# Autodesk Inventor assembly: Assembly2
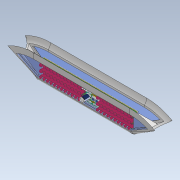
[picture p0: Inventor's stored thumbnail of the model, 180x180]
Saved by Autodesk Inventor 2021 (Build 250183000, 183)
## iProperties
Created: 2020-10-01
Part Number: Assembly2
Document SubType Name: Assembly
Designer: capta
Author: capta
## Documents named in this file (5)
- C:\Users\capta\OneDrive - Lehigh University\Formula SAE\Tractive Light\Assembly2.iam
- C:\Users\capta\OneDrive - Lehigh University\Formula SAE\Tractive Light\Tractive Light Enclosure 3.0.ipt
- C:\Users\capta\OneDrive - Lehigh University\Formula SAE\Tractive Light\Mount CAD\pcd stand in.ipt
- C:\Users\capta\OneDrive - Lehigh University\Formula SAE\Tractive Light\acrlyc 2.0.ipt
- C:\Users\capta\OneDrive - Lehigh University\Formula SAE\Tractive Light\PCB Assembly\Tractive PCB.iam
## Components (5 placed, 4 different names)
1. Tractive Light Enclosure 3.0:1 — Mate:1, Mate:2, Mate:3, Mate:4, Mate:5, Mate:6, Mate:7, Mate:8, Mate:9, Mate:10, Mate:11, Mate:12
2. pcd stand in:1 — Mate:1, Mate:2, Mate:3
3. acrlyc 2.0:1 — Mate:4, Mate:5, Mate:6
4. acrlyc 2.0:2 — Mate:7, Mate:8, Mate:9
5. Tractive PCB:1 [sub-assembly] — Mate:10, Mate:11, Mate:12
## Relationships (14: Mate 12, Flush 2)
- Mate:1: Tractive Light Enclosure 3.0:1 ↔ pcd stand in:1
- Mate:2 (0.381 mm): Tractive Light Enclosure 3.0:1 ↔ pcd stand in:1
- Mate:3 (0.0762 mm): Tractive Light Enclosure 3.0:1 ↔ pcd stand in:1
- Mate:4: Tractive Light Enclosure 3.0:1 ↔ acrlyc 2.0:1
- Mate:5: Tractive Light Enclosure 3.0:1 ↔ acrlyc 2.0:1
- Mate:6: Tractive Light Enclosure 3.0:1 ↔ acrlyc 2.0:1
- Mate:7: Tractive Light Enclosure 3.0:1 ↔ acrlyc 2.0:2
- Mate:8: Tractive Light Enclosure 3.0:1 ↔ acrlyc 2.0:2
- Mate:9: Tractive Light Enclosure 3.0:1 ↔ acrlyc 2.0:2
- Flush:1 (96.407 mm)
- Flush:2 (-106.7067 mm)
- Mate:10: Tractive Light Enclosure 3.0:1 ↔ Tractive PCB:1
- Mate:11: Tractive Light Enclosure 3.0:1 ↔ Tractive PCB:1
- Mate:12 (0.0889 mm): Tractive Light Enclosure 3.0:1 ↔ Tractive PCB:1
